# Autodesk Inventor assembly: Blade-2
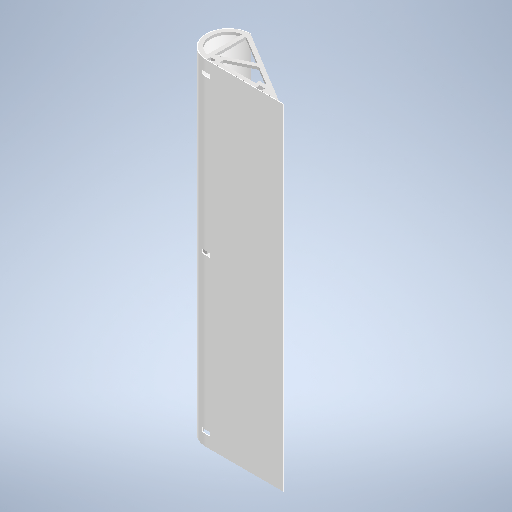
[picture p0: Inventor's stored thumbnail of the model, 512x512]
Saved by Autodesk Inventor 2025.1 (Build 291241000, 241)
## iProperties
Created: 2025-01-28
Part Number: Blade-2
Document SubType Name: Assembly
Designer: Dimas Arif
Author: Dimas Arif
## Documents named in this file (4)
- C:\Users\Dimas Arif\Documents\Inventor\Project-81\Blade-2.iam
- C:\Users\Dimas Arif\Documents\Inventor\Project-81\Balde.ipt
- C:\Users\Dimas Arif\Documents\Inventor\Project-81\F1.ipt
- C:\Users\Dimas Arif\Documents\Inventor\Project-81\P1.ipt
## Components (5 placed, 3 different names)
1. F1:1 — Mate:1, Mate:2, Flush:2
2. Balde:1 — Flush:1, Flush:3, Flush:4
3. P1:1 — Flush:1, Mate:1, Mate:2, Flush:2
4. P1:2
5. P1:3
## Component patterns: (3 elements, first: P1:1)
## Relationships (8: Flush 4, Mate 4)
- Flush:1: Balde:1 ↔ P1:1
- Mate:1: F1:1 ↔ P1:1
- Mate:2: F1:1 ↔ P1:1
- Flush:2: F1:1 ↔ P1:1
- Flush:3 (500 mm): Balde:1
- Flush:4 (-194 mm): Balde:1
- Mate:3
- Mate:4
